# Autodesk Inventor assembly: SSR-40 DA Small P W S
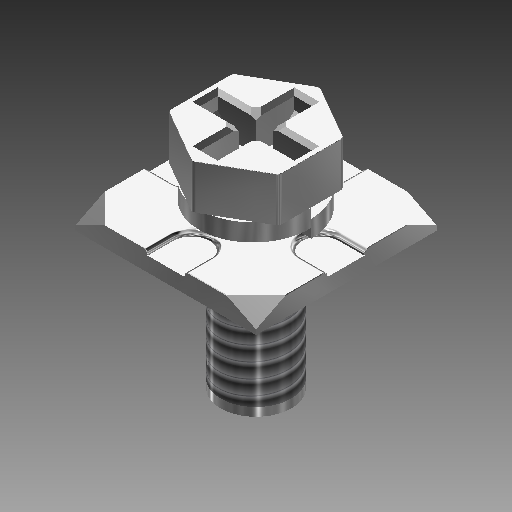
[picture p0: Inventor's stored thumbnail of the model, 512x512]
Saved by Autodesk Inventor 2019 (Build 230136000, 136)
## iProperties
Created: 2014-11-01
Part Number: SSR-40 DA Small P W S
Document SubType Name: Assembly
Designer: Tyler
Author: Tyler
## Documents named in this file (4)
- C:\Users\Ax\Google Drive\Inventor\Library\SSR-40 DA Small P W S.iam
- C:\Users\Ax\Google Drive\Inventor\Library\SSR-40 DA Screw.ipt
- C:\Users\Ax\Google Drive\Inventor\Library\SSR-40 DA Lock Washer.ipt
- C:\Users\Ax\Google Drive\Inventor\Library\SSR-40 DA Small Plate.ipt
## Components (3 placed, 3 different names)
1. SSR-40 DA Screw:1 — Mate:2, Mate:3
2. SSR-40 DA Lock Washer:1 — Mate:2
3. SSR-40 DA Small Plate:1 — Mate:3
## Relationships (2: Mate 2)
- Mate:2: SSR-40 DA Screw:1 ↔ SSR-40 DA Lock Washer:1
- Mate:3: SSR-40 DA Screw:1 ↔ SSR-40 DA Small Plate:1
